# Autodesk Inventor assembly: Assembly3
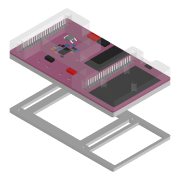
[picture p0: Inventor's stored thumbnail of the model, 180x180]
Saved by Autodesk Inventor 2020 (Build 240168000, 168)
## iProperties
Created: 2021-07-01
Part Number: Assembly3
Document SubType Name: Assembly
Designer: ferrerx
Author: ferrerx
## Documents named in this file (5)
- C:\Users\ferrerx\Desktop\Sport analyzer\Sport Analyzer 1.0.1\Mechanical\Assembly3.iam
- C:\Users\ferrerx\Desktop\Sport analyzer\Sport Analyzer 1.0.1\Mechanical\Sport Analyzer 1.0.1 PCB .iam
- C:\Users\ferrerx\Desktop\Sport analyzer\Sport Analyzer 1.0.1\Mechanical\Bottom PMMA.ipt
- C:\Users\ferrerx\Desktop\Sport analyzer\Sport Analyzer 1.0.1\Mechanical\Middle PMMA.ipt
- C:\Users\ferrerx\Desktop\Sport analyzer\Sport Analyzer 1.0.1\Mechanical\Top PMMA.ipt
## Components (4 placed, 4 different names)
1. Sport Analyzer 1.0.1 PCB :1 [sub-assembly] — Mate:1, Flush:1, Flush:2, Mate:2
2. Bottom PMMA:1 — Mate:1, Flush:1, Flush:2, Flush:3, Flush:4
3. Middle PMMA:1 — Flush:3, Mate:2, Flush:4, Flush:5, Flush:6
4. Top PMMA:1 — Flush:5, Flush:6
## Relationships (8: Flush 6, Mate 2)
- Mate:1: Sport Analyzer 1.0.1 PCB :1 ↔ Bottom PMMA:1
- Flush:1: Sport Analyzer 1.0.1 PCB :1 ↔ Bottom PMMA:1
- Flush:2: Sport Analyzer 1.0.1 PCB :1 ↔ Bottom PMMA:1
- Flush:3: Bottom PMMA:1 ↔ Middle PMMA:1
- Mate:2: Sport Analyzer 1.0.1 PCB :1 ↔ Middle PMMA:1
- Flush:4: Bottom PMMA:1 ↔ Middle PMMA:1
- Flush:5: Middle PMMA:1 ↔ Top PMMA:1
- Flush:6: Middle PMMA:1 ↔ Top PMMA:1
